# Autodesk Inventor assembly: manipulator
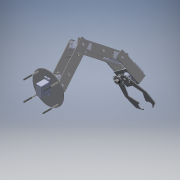
[picture p0: Inventor's stored thumbnail of the model, 180x180]
Saved by Autodesk Inventor 2017.3 (Build 213256000, 256)
## iProperties
Part Number: manipulator
Material: Ogólny
Document SubType Name: Assembly
Designer: legox
Author: legox
## iProperties of the stored document Servo-MG90S.ipt
Created: 2017-09-26
Part Number: Servo-MG90S
Material: Ogólny
Document SubType Name: Modeling
Designer: legox
Density: 1 g/cm^3
Appearance: Domyślna
Sending System: SolidWorks 2017
Last Author: Lynx
Last Saved: 2017-09-26
Author: legox
## Documents named in this file (18)
- **C:\Users\legox\Documents\Inventor\Content Center Files\manipulator\manipulator.iam*LocalDocs*x1hpyqbugUmd5ui4p1ii0ced2Nh*Servo-MG90S.ipt
- C:\Users\legox\Documents\Inventor\Content Center Files\manipulator\manipulator.iam
- C:\Users\legox\Documents\Inventor\Content Center Files\manipulator\podstawa1.ipt
- C:\Users\legox\Documents\Inventor\Content Center Files\manipulator\podstawa2.ipt
- C:\Users\legox\Documents\Inventor\Content Center Files\manipulator\mocowanie do podstawy2.ipt
- C:\Users\legox\Documents\Inventor\Content Center Files\manipulator\ramie2.ipt
- C:\Users\legox\Documents\Inventor\Content Center Files\manipulator\ramie1a.ipt
- C:\Users\legox\Documents\Inventor\Content Center Files\manipulator\ramie3.ipt
- C:\Users\legox\Documents\Inventor\Content Center Files\manipulator\mocowanie ostatniego serwa.ipt
- C:\Users\legox\Documents\Inventor\Content Center Files\manipulator\efektor zebatka1.ipt
- C:\Users\legox\Documents\Inventor\Content Center Files\manipulator\efektor szczypce1.ipt
- C:\Users\legox\Documents\Inventor\Content Center Files\R2017\pl-PL\ANSI B 18.2.4.1 M(1)\ANSI B 18.2.4.1 M - M3 x 0,5Style 1.ipt
- C:\Users\legox\Documents\Inventor\Content Center Files\R2017\pl-PL\U 2494(1)\Unbrako - M3 x  25(6).ipt
- C:\Users\legox\Documents\Inventor\Content Center Files\R2017\pl-PL\U 2494(1)\Unbrako - M3 x  35(6).ipt
- C:\Users\legox\Documents\Inventor\Content Center Files\R2017\pl-PL\U 2494(1)\Unbrako - M5 x  30(6).ipt
- C:\Users\legox\Documents\Inventor\Content Center Files\R2017\pl-PL\ANSI B 18.2.4.1 M(1)\ANSI B 18.2.4.1 M - M5 x 0,8Style 1.ipt
- C:\Users\legox\Documents\Inventor\Content Center Files\manipulator\dystansik.ipt
- C:\Users\legox\Documents\Inventor\Content Center Files\manipulator\Servo-MG90S.SLDPRT
## Components (39 placed, 16 different names)
1. podstawa1:1 — Zestawiający:1, Zestawiający:2, Zestawiający:3, Kąt:7, Kąt:8, Kąt:9, Zestawiający:97, Zestawiający:98, Zestawiający:99, Zestawiający:100, Styczny:23, Styczny:24, Styczny:25, Styczny:26
2. podstawa2:1 — Zestawiający:52, Zestawiający:55, Zestawiający:56, Styczny:1, Styczny:2, Styczny:3
3. Servo-MG90S:1 — Zestawiający:1, Zestawiający:2, Zestawiający:3, Zestawiający:53, Zestawiający:55
4. Servo-MG90S:2 — Zestawiający:9, Zestawiający:18, Zestawiający:34, Równoległy:4, Zestawiający:37, Zestawiający:56, Styczny:1, Styczny:2, Styczny:3, Styczny:4, Styczny:5, Styczny:6
5. mocowanie do podstawy2:1 — Zestawiający:9, Zestawiający:46, Zestawiający:49, Styczny:4, Styczny:5, Styczny:6, Zestawiający:93, Zestawiający:94, Zestawiający:95, Zestawiający:96, Styczny:19, Styczny:20, Styczny:21, Styczny:22
6. Servo-MG90S:3 — Zestawiający:20, Zestawiający:22, Równoległy:3, Zestawiający:23, Zestawiający:24, Zestawiający:25, Zestawiający:26, Zestawiający:35, Równoległy:5
7. ramie2:1 — Równoległy:3, Zestawiający:25, Zestawiający:26, Styczny:7, Zestawiający:84, Zestawiający:89
8. ramie2:2 — Zestawiający:22, Zestawiający:23, Zestawiający:24, Zestawiający:27, Zestawiający:28, Zestawiający:29, Kąt:8, Zestawiający:81
9. Servo-MG90S:4 — Zestawiający:27, Zestawiający:28, Zestawiający:29, Równoległy:14, Zestawiający:78
10. ramie1a:1 — Zestawiający:32, Zestawiający:33, Zestawiający:37, Zestawiający:38, Zestawiający:39, Zestawiający:85, Zestawiający:86, Zestawiający:87, Zestawiający:88
11. ramie1a:2 — Zestawiający:30, Zestawiający:31, Równoległy:4, Równoległy:5, Kąt:7, Zestawiający:82, Zestawiający:83, Styczny:8, Styczny:9
12. ramie3:1 — Równoległy:7, Równoległy:8, Równoległy:9, Zestawiający:60, Kąt:5, Kąt:9
13. ramie3:2 — Równoległy:7, Kąt:10, Równoległy:12, Zestawiający:77, Równoległy:13, Równoległy:14, Zestawiający:79
14. Servo-MG90S:5 — Zestawiający:61, Zestawiający:62, Zestawiający:63, Zestawiający:65, Równoległy:11
15. mocowanie ostatniego serwa:1 — Równoległy:8, Równoległy:9, Zestawiający:60, Zestawiający:61, Zestawiający:62, Zestawiający:63, Zestawiający:66, Kąt:3, Kąt:4, Równoległy:12, Zestawiający:77, Równoległy:13, Zestawiający:90
16. efektor zebatka1:1 — Zestawiający:64, Równoległy:10, Równoległy:11, Kąt:3, Zestawiający:76
17. efektor zebatka1:2 — Zestawiający:68, Równoległy:10, Kąt:4, Zestawiający:75, Zestawiający:91
18. efektor szczypce1:1 — Zestawiający:70, Kąt:5, Zestawiający:76
19. efektor szczypce1:2 — Zestawiający:73, Kąt:10, Zestawiający:75, Styczny:16, Zestawiający:92
20. Unbrako Śruba z łbem walcowym z gniazdem sześciokątnym - Metryczny M3 x 25:1 — Zestawiający:81, Styczny:7, Styczny:10, Styczny:15
21. Unbrako Śruba z łbem walcowym z gniazdem sześciokątnym - Metryczny M3 x 35:1 — Zestawiający:82, Styczny:9, Styczny:12, Styczny:14
22. Unbrako Śruba z łbem walcowym z gniazdem sześciokątnym - Metryczny M3 x 35:2 — Zestawiający:83, Styczny:8, Styczny:11, Styczny:13
23. Nakrętka Metryczny M3 x 0,5:1 — Zestawiający:85, Styczny:11
24. Nakrętka Metryczny M3 x 0,5:2 — Zestawiający:86, Styczny:12
25. Nakrętka Metryczny M3 x 0,5:3 — Zestawiający:87, Styczny:13
26. Nakrętka Metryczny M3 x 0,5:4 — Zestawiający:84, Styczny:10
27. Nakrętka Metryczny M3 x 0,5:5 — Zestawiający:88, Styczny:14
28. Nakrętka Metryczny M3 x 0,5:6 — Zestawiający:89, Styczny:15
29. Unbrako Śruba z łbem walcowym z gniazdem sześciokątnym - Metryczny M5 x 30:1 — Zestawiający:90, Styczny:16, Styczny:17, Styczny:18
30. Nakrętka Metryczny M5 x 0,8:1 — Zestawiający:91, Styczny:17
31. dystansik:1 — Styczny:18, Zestawiający:92
32. Unbrako Śruba z łbem walcowym z gniazdem sześciokątnym - Metryczny M3 x 25:2 — Zestawiający:93, Styczny:20
33. Unbrako Śruba z łbem walcowym z gniazdem sześciokątnym - Metryczny M3 x 25:3 — Zestawiający:94, Styczny:22
34. Unbrako Śruba z łbem walcowym z gniazdem sześciokątnym - Metryczny M3 x 25:4 — Zestawiający:95, Styczny:19
35. Unbrako Śruba z łbem walcowym z gniazdem sześciokątnym - Metryczny M3 x 25:5 — Zestawiający:96, Styczny:21
36. Unbrako Śruba z łbem walcowym z gniazdem sześciokątnym - Metryczny M3 x 35:3 — Zestawiający:100, Styczny:25
37. Unbrako Śruba z łbem walcowym z gniazdem sześciokątnym - Metryczny M3 x 35:4 — Zestawiający:99, Styczny:23
38. Unbrako Śruba z łbem walcowym z gniazdem sześciokątnym - Metryczny M3 x 35:5 — Zestawiający:98, Styczny:24
39. Unbrako Śruba z łbem walcowym z gniazdem sześciokątnym - Metryczny M3 x 35:6 — Zestawiający:97, Styczny:26
## Relationships (121: Mate 77, Tangent 26, Flush 11, Angle 7)
- Zestawiający:1 [Mate]: podstawa1:1 ↔ Servo-MG90S:1
- Zestawiający:2 [Mate]: podstawa1:1 ↔ Servo-MG90S:1
- Zestawiający:3 [Mate]: podstawa1:1 ↔ Servo-MG90S:1
- Zestawiający:9 [Mate]: Servo-MG90S:2 ↔ mocowanie do podstawy2:1
- Zestawiający:16 [Mate]
- Zestawiający:17 [Mate]
- Zestawiający:18 [Mate]: Servo-MG90S:2
- Zestawiający:19 [Mate]
- Zestawiający:20 [Mate]: Servo-MG90S:3
- Zestawiający:21 [Mate]
- Zestawiający:22 [Mate]: Servo-MG90S:3 ↔ ramie2:2
- Równoległy:3 [Flush]: Servo-MG90S:3 ↔ ramie2:1
- Zestawiający:23 [Mate]: Servo-MG90S:3 ↔ ramie2:2
- Zestawiający:24 [Mate]: Servo-MG90S:3 ↔ ramie2:2
- Zestawiający:25 [Mate]: Servo-MG90S:3 ↔ ramie2:1
- Zestawiający:26 [Mate]: Servo-MG90S:3 ↔ ramie2:1
- Zestawiający:27 [Mate]: ramie2:2 ↔ Servo-MG90S:4
- Zestawiający:28 [Mate]: ramie2:2 ↔ Servo-MG90S:4
- Zestawiający:29 [Mate]: ramie2:2 ↔ Servo-MG90S:4
- Zestawiający:30 [Mate]: ramie1a:2
- Zestawiający:31 [Mate]: ramie1a:2
- Zestawiający:32 [Mate]: ramie1a:1
- Zestawiający:33 [Mate]: ramie1a:1
- Zestawiający:34 [Mate]: Servo-MG90S:2
- Zestawiający:35 [Mate]: Servo-MG90S:3
- Zestawiający:36 [Mate]
- Równoległy:4 [Flush]: Servo-MG90S:2 ↔ ramie1a:2
- Zestawiający:37 [Mate]: Servo-MG90S:2 ↔ ramie1a:1
- Zestawiający:38 [Mate]: ramie1a:1
- Zestawiający:39 [Mate]: ramie1a:1
- Zestawiający:40 [Mate]
- Równoległy:5 [Flush]: Servo-MG90S:3 ↔ ramie1a:2
- Zestawiający:46 [Mate]: mocowanie do podstawy2:1
- Zestawiający:48 [Mate]
- Zestawiający:49 [Mate]: mocowanie do podstawy2:1
- Zestawiający:51 [Mate]
- Zestawiający:52 [Mate]: podstawa2:1
- Zestawiający:53 [Mate]: Servo-MG90S:1
- Zestawiający:54 [Mate]
- Zestawiający:55 [Mate]: podstawa2:1 ↔ Servo-MG90S:1
- Zestawiający:56 [Mate]: podstawa2:1 ↔ Servo-MG90S:2
- Styczny:1 [Tangent]: podstawa2:1 ↔ Servo-MG90S:2
- Styczny:2 [Tangent]: podstawa2:1 ↔ Servo-MG90S:2
- Styczny:3 [Tangent]: podstawa2:1 ↔ Servo-MG90S:2
- Styczny:4 [Tangent]: Servo-MG90S:2 ↔ mocowanie do podstawy2:1
- Styczny:5 [Tangent]: Servo-MG90S:2 ↔ mocowanie do podstawy2:1
- Styczny:6 [Tangent]: Servo-MG90S:2 ↔ mocowanie do podstawy2:1
- Równoległy:7 [Flush]: ramie3:1 ↔ ramie3:2
- Równoległy:8 [Flush]: ramie3:1 ↔ mocowanie ostatniego serwa:1
- Równoległy:9 [Flush]: ramie3:1 ↔ mocowanie ostatniego serwa:1
- Zestawiający:60 [Mate]: ramie3:1 ↔ mocowanie ostatniego serwa:1
- Zestawiający:61 [Mate]: Servo-MG90S:5 ↔ mocowanie ostatniego serwa:1
- Zestawiający:62 [Mate]: Servo-MG90S:5 ↔ mocowanie ostatniego serwa:1
- Zestawiający:63 [Mate]: Servo-MG90S:5 ↔ mocowanie ostatniego serwa:1
- Zestawiający:64 [Mate]: efektor zebatka1:1
- Zestawiający:65 [Mate]: Servo-MG90S:5
- Zestawiający:66 [Mate]: mocowanie ostatniego serwa:1
- Zestawiający:67 [Mate]
- Zestawiający:68 [Mate]: efektor zebatka1:2
- Równoległy:10 [Flush]: efektor zebatka1:1 ↔ efektor zebatka1:2
- Równoległy:11 [Flush]: Servo-MG90S:5 ↔ efektor zebatka1:1
- Zestawiający:70 [Mate]: efektor szczypce1:1
- Zestawiający:71 [Mate]
- Zestawiający:73 [Mate]: efektor szczypce1:2
- Zestawiający:74 [Mate]
- Kąt:3 [Angle] (0 deg): mocowanie ostatniego serwa:1 ↔ efektor zebatka1:1
- Kąt:4 [Angle] (15 deg): mocowanie ostatniego serwa:1 ↔ efektor zebatka1:2
- Kąt:5 [Angle] (-20 deg): ramie3:1 ↔ efektor szczypce1:1
- Kąt:7 [Angle] (120 deg): podstawa1:1 ↔ ramie1a:2
- Kąt:8 [Angle] (230 deg): podstawa1:1 ↔ ramie2:2
- Kąt:9 [Angle] (20 deg): podstawa1:1 ↔ ramie3:1
- Kąt:10 [Angle] (20 deg): ramie3:2 ↔ efektor szczypce1:2
- Zestawiający:75 [Mate]: efektor zebatka1:2 ↔ efektor szczypce1:2
- Zestawiający:76 [Mate]: efektor zebatka1:1 ↔ efektor szczypce1:1
- Równoległy:12 [Flush]: ramie3:2 ↔ mocowanie ostatniego serwa:1
- Zestawiający:77 [Mate]: ramie3:2 ↔ mocowanie ostatniego serwa:1
- Równoległy:13 [Flush]: ramie3:2 ↔ mocowanie ostatniego serwa:1
- Równoległy:14 [Flush]: Servo-MG90S:4 ↔ ramie3:2
- Zestawiający:78 [Mate]: Servo-MG90S:4
- Zestawiający:79 [Mate]: ramie3:2
- Zestawiający:80 [Mate]
- Zestawiający:81 [Mate]: ramie2:2 ↔ Unbrako Śruba z łbem walcowym z gniazdem sześciokątnym - Metryczny M3 x 25:1
- Styczny:7 [Tangent]: ramie2:1 ↔ Unbrako Śruba z łbem walcowym z gniazdem sześciokątnym - Metryczny M3 x 25:1
- Zestawiający:82 [Mate]: ramie1a:2 ↔ Unbrako Śruba z łbem walcowym z gniazdem sześciokątnym - Metryczny M3 x 35:1
- Zestawiający:83 [Mate]: ramie1a:2 ↔ Unbrako Śruba z łbem walcowym z gniazdem sześciokątnym - Metryczny M3 x 35:2
- Styczny:8 [Tangent]: ramie1a:2 ↔ Unbrako Śruba z łbem walcowym z gniazdem sześciokątnym - Metryczny M3 x 35:2
- Styczny:9 [Tangent]: ramie1a:2 ↔ Unbrako Śruba z łbem walcowym z gniazdem sześciokątnym - Metryczny M3 x 35:1
- Zestawiający:84 [Mate]: ramie2:1 ↔ Nakrętka Metryczny M3 x 0,5:4
- Zestawiający:85 [Mate]: ramie1a:1 ↔ Nakrętka Metryczny M3 x 0,5:1
- Zestawiający:86 [Mate]: ramie1a:1 ↔ Nakrętka Metryczny M3 x 0,5:2
- Zestawiający:87 [Mate]: ramie1a:1 ↔ Nakrętka Metryczny M3 x 0,5:3
- Zestawiający:88 [Mate]: ramie1a:1 ↔ Nakrętka Metryczny M3 x 0,5:5
- Zestawiający:89 [Mate]: ramie2:1 ↔ Nakrętka Metryczny M3 x 0,5:6
- Styczny:10 [Tangent]: Unbrako Śruba z łbem walcowym z gniazdem sześciokątnym - Metryczny M3 x 25:1 ↔ Nakrętka Metryczny M3 x 0,5:4
- Styczny:11 [Tangent]: Unbrako Śruba z łbem walcowym z gniazdem sześciokątnym - Metryczny M3 x 35:2 ↔ Nakrętka Metryczny M3 x 0,5:1
- Styczny:12 [Tangent]: Unbrako Śruba z łbem walcowym z gniazdem sześciokątnym - Metryczny M3 x 35:1 ↔ Nakrętka Metryczny M3 x 0,5:2
- Styczny:13 [Tangent]: Unbrako Śruba z łbem walcowym z gniazdem sześciokątnym - Metryczny M3 x 35:2 ↔ Nakrętka Metryczny M3 x 0,5:3
- Styczny:14 [Tangent]: Unbrako Śruba z łbem walcowym z gniazdem sześciokątnym - Metryczny M3 x 35:1 ↔ Nakrętka Metryczny M3 x 0,5:5
- Styczny:15 [Tangent]: Unbrako Śruba z łbem walcowym z gniazdem sześciokątnym - Metryczny M3 x 25:1 ↔ Nakrętka Metryczny M3 x 0,5:6
- Zestawiający:90 [Mate]: mocowanie ostatniego serwa:1 ↔ Unbrako Śruba z łbem walcowym z gniazdem sześciokątnym - Metryczny M5 x 30:1
- Styczny:16 [Tangent]: efektor szczypce1:2 ↔ Unbrako Śruba z łbem walcowym z gniazdem sześciokątnym - Metryczny M5 x 30:1
- Zestawiający:91 [Mate]: efektor zebatka1:2 ↔ Nakrętka Metryczny M5 x 0,8:1
- Styczny:17 [Tangent]: Unbrako Śruba z łbem walcowym z gniazdem sześciokątnym - Metryczny M5 x 30:1 ↔ Nakrętka Metryczny M5 x 0,8:1
- Styczny:18 [Tangent]: Unbrako Śruba z łbem walcowym z gniazdem sześciokątnym - Metryczny M5 x 30:1 ↔ dystansik:1
- Zestawiający:92 [Mate]: efektor szczypce1:2 ↔ dystansik:1
- Zestawiający:93 [Mate]: mocowanie do podstawy2:1 ↔ Unbrako Śruba z łbem walcowym z gniazdem sześciokątnym - Metryczny M3 x 25:2
- Zestawiający:94 [Mate]: mocowanie do podstawy2:1 ↔ Unbrako Śruba z łbem walcowym z gniazdem sześciokątnym - Metryczny M3 x 25:3
- Zestawiający:95 [Mate]: mocowanie do podstawy2:1 ↔ Unbrako Śruba z łbem walcowym z gniazdem sześciokątnym - Metryczny M3 x 25:4
- Zestawiający:96 [Mate]: mocowanie do podstawy2:1 ↔ Unbrako Śruba z łbem walcowym z gniazdem sześciokątnym - Metryczny M3 x 25:5
- Styczny:19 [Tangent]: mocowanie do podstawy2:1 ↔ Unbrako Śruba z łbem walcowym z gniazdem sześciokątnym - Metryczny M3 x 25:4
- Styczny:20 [Tangent]: mocowanie do podstawy2:1 ↔ Unbrako Śruba z łbem walcowym z gniazdem sześciokątnym - Metryczny M3 x 25:2
- Styczny:21 [Tangent]: mocowanie do podstawy2:1 ↔ Unbrako Śruba z łbem walcowym z gniazdem sześciokątnym - Metryczny M3 x 25:5
- Styczny:22 [Tangent]: mocowanie do podstawy2:1 ↔ Unbrako Śruba z łbem walcowym z gniazdem sześciokątnym - Metryczny M3 x 25:3
- Zestawiający:97 [Mate]: podstawa1:1 ↔ Unbrako Śruba z łbem walcowym z gniazdem sześciokątnym - Metryczny M3 x 35:6
- Zestawiający:98 [Mate]: podstawa1:1 ↔ Unbrako Śruba z łbem walcowym z gniazdem sześciokątnym - Metryczny M3 x 35:5
- Zestawiający:99 [Mate]: podstawa1:1 ↔ Unbrako Śruba z łbem walcowym z gniazdem sześciokątnym - Metryczny M3 x 35:4
- Zestawiający:100 [Mate]: podstawa1:1 ↔ Unbrako Śruba z łbem walcowym z gniazdem sześciokątnym - Metryczny M3 x 35:3
- Styczny:23 [Tangent]: podstawa1:1 ↔ Unbrako Śruba z łbem walcowym z gniazdem sześciokątnym - Metryczny M3 x 35:4
- Styczny:24 [Tangent]: podstawa1:1 ↔ Unbrako Śruba z łbem walcowym z gniazdem sześciokątnym - Metryczny M3 x 35:5
- Styczny:25 [Tangent]: podstawa1:1 ↔ Unbrako Śruba z łbem walcowym z gniazdem sześciokątnym - Metryczny M3 x 35:3
- Styczny:26 [Tangent]: podstawa1:1 ↔ Unbrako Śruba z łbem walcowym z gniazdem sześciokątnym - Metryczny M3 x 35:6
